# Autodesk Inventor assembly: WinderAssembly
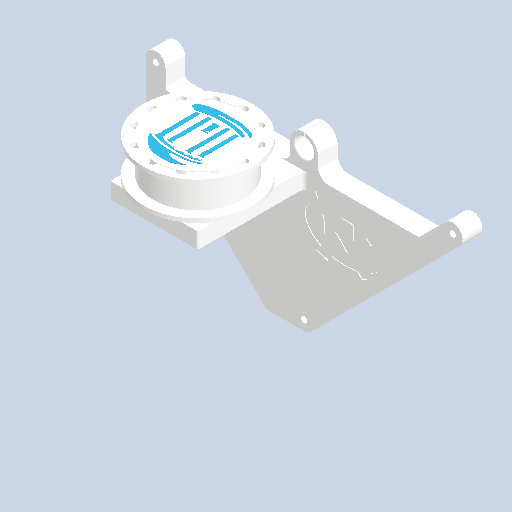
[picture p0: Inventor's stored thumbnail of the model, 512x512]
Saved by Autodesk Inventor 2022 (Build 260153000, 153)
## iProperties
Created: 2020-03-15
Part Number: WinderAssembly
Document SubType Name: Assembly
Designer: elmar
Author: elmar
## Documents named in this file (4)
- C:\repo\FourWireBraidingMachine\InventorFiles\WinderAssembly.iam
- C:\repo\FourWireBraidingMachine\InventorFiles\WinderSpool.ipt
- C:\repo\FourWireBraidingMachine\InventorFiles\WinderBracket.ipt
- C:\repo\FourWireBraidingMachine\InventorFiles\ShaftPlate.ipt
## Components (3 placed, 3 different names)
1. WinderSpool:1 — Insert:1
2. WinderBracket:1 — Insert:1, Insert:2
3. ShaftPlate:1 — Insert:2
## Relationships (2: Insert 2)
- Insert:1 (1 mm): WinderSpool:1 ↔ WinderBracket:1
- Insert:2 (0.5 mm): WinderBracket:1 ↔ ShaftPlate:1
